# Autodesk Inventor assembly: Assembly base
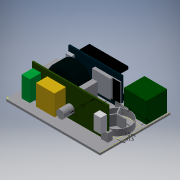
[picture p0: Inventor's stored thumbnail of the model, 180x180]
Saved by Autodesk Inventor 2019 (Build 230136000, 136)
## iProperties
Created: 2022-02-04
Part Number: Assembly base
Document SubType Name: Assembly
Designer: josec
Author: josec
## Documents named in this file (6)
- C:\Users\josec\Documents\Inventor\Enchufe\Assembly base.iam
- C:\Users\josec\Documents\Inventor\Enchufe\base.ipt
- C:\Users\josec\Documents\Inventor\Enchufe\PZEM-00ET.ipt
- C:\Users\josec\Documents\Inventor\Enchufe\ESP32.ipt
- C:\Users\josec\Documents\Inventor\Enchufe\coil.ipt
- C:\Users\josec\Documents\Inventor\Enchufe\power supply.ipt
## Components (5 placed, 5 different names)
1. base:1 — Mate:1, Mate:2, Mate:3, Mate:4, Mate:5, Mate:6, Rotational:1, Mate:7, Mate:8, Mate:9
2. PZEM-00ET:1 — Mate:1, Mate:2, Mate:3
3. ESP32:1 — Mate:4, Mate:5, Mate:6
4. coil:1 — Rotational:1
5. power supply:1 — Mate:7, Mate:8, Mate:9
## Relationships (10: Mate 9, RevoluteJoint 1)
- Mate:1: base:1 ↔ PZEM-00ET:1
- Mate:2: base:1 ↔ PZEM-00ET:1
- Mate:3: base:1 ↔ PZEM-00ET:1
- Mate:4: base:1 ↔ ESP32:1
- Mate:5: base:1 ↔ ESP32:1
- Mate:6: base:1 ↔ ESP32:1
- Rotational:1 [RevoluteJoint]: base:1 ↔ coil:1
- Mate:7: base:1 ↔ power supply:1
- Mate:8: base:1 ↔ power supply:1
- Mate:9: base:1 ↔ power supply:1
